# Autodesk Inventor assembly: testbracket
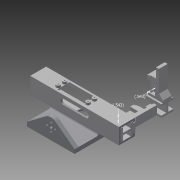
[picture p0: Inventor's stored thumbnail of the model, 180x180]
Saved by Autodesk Inventor 2015 (Build 190159000, 159)
## iProperties
Created: 2014-12-16
Part Number: testbracket
Document SubType Name: Assembly
Designer: Rene
Author: Rene
## Documents named in this file (3)
- D:\Rene\Documents\CSE462\physical\Finals\testbracket.iam
- D:\Rene\Documents\CSE462\physical\Finals\newbracket.ipt
- D:\Rene\Documents\CSE462\physical\Finals\mod_gripper.ipt
## Components (3 placed, 2 different names)
1. newbracket:1 — Mate:1, Mate:2
2. mod_gripper:1 — Mate:1, Mate:2
3. mod_gripper:2
## Relationships (2: Mate 2)
- Mate:1: newbracket:1 ↔ mod_gripper:1
- Mate:2 (0.508 mm): newbracket:1 ↔ mod_gripper:1
